# Autodesk Inventor assembly: 20-J2
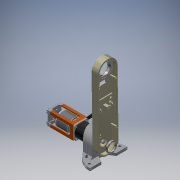
[picture p0: Inventor's stored thumbnail of the model, 180x180]
Saved by Autodesk Inventor 2018 (Build 220112000, 112)
## iProperties
Created: 2020-01-14
Part Number: 20-J2
Document SubType Name: Assembly
Designer: Bunny320
Author: Bunny320
## Documents named in this file (10)
- C:\Users\Bunny320\Desktop\sechs\4-CAD\30-J3.iam
- C:\Users\Bunny320\Desktop\sechs\4-CAD\201-flange-with motor.ipt
- C:\Users\Bunny320\Desktop\sechs\4-CAD\standardParts\61807-2RS1\61807-2RS1.iam
- C:\Users\Bunny320\Desktop\sechs\4-CAD\motor unit.iam
- C:\Users\Bunny320\Desktop\sechs\4-CAD\303-link right.ipt
- C:\Users\Bunny320\Desktop\sechs\4-CAD\generated\J3_belt.iam
- C:\Users\Bunny320\Desktop\sechs\4-CAD\standardParts\61705-2RZ\W 61705-2RZ.iam
- C:\Users\Bunny320\Desktop\sechs\4-CAD\standardParts\W 638_3-2Z\W 638_3-2Z.iam
- C:\Users\Bunny320\Documents\Inventor\Content Center Files\R2018\en-US\ISO 10642(2)\ISO 10642  - M4  x  20.ipt
- C:\Users\Bunny320\Documents\Inventor\Content Center Files\R2018\en-US\ISO 4762(1)\DIN EN ISO 4762 - M3 x 12.ipt
## Components (15 placed, 9 different names)
1. 201-flange-with motor:1 — Flush:1, Flush:2, Flush:3, Mate:3, Mate:4, Mate:7, Mate:8, Mate:9, Mate:22, Mate:23, Mate:24, Mate:25
2. 61807-2RS1:1 [sub-assembly] — Mate:3, Mate:4, Mate:10, Mate:11
3. 61807-2RS1:2 [sub-assembly] — Mate:12, Mate:13
4. motor unit:1 [sub-assembly] — Mate:7, Mate:8, Mate:9, Mate:14
5. 303-link right:1 — Mate:10, Mate:11, Mate:12, Mate:13, Flush:4, Mate:17, Mate:18, Mate:19, Mate:20, Mate:21, Mate:26, Mate:32
6. J3_belt:1 [sub-assembly] — Flush:4, Mate:14, Mate:15, Mate:16, Mate:17
7. W 61705-2RZ:1 [sub-assembly] — Mate:15, Mate:16
8. W 638_3-2Z:1 [sub-assembly] — Mate:18, Mate:21, Mate:27, Mate:33
9. W 638_3-2Z:2 [sub-assembly] — Mate:19, Mate:20
10. DIN EN ISO 10642 M4  x  20:1 — Mate:22
11. DIN EN ISO 10642 M4  x  20:2 — Mate:23
12. DIN EN ISO 10642 M4  x  20:3 — Mate:24
13. DIN EN ISO 10642 M4  x  20:4 — Mate:25
14. DIN EN ISO 4762 M3 x 12:1 — Mate:26, Mate:27
15. DIN EN ISO 4762 M3 x 12:4 — Mate:32, Mate:33
## Relationships (29: Mate 25, Flush 4)
- Flush:1: 201-flange-with motor:1
- Flush:2: 201-flange-with motor:1
- Flush:3: 201-flange-with motor:1
- Mate:3: 201-flange-with motor:1 ↔ 61807-2RS1:1
- Mate:4: 201-flange-with motor:1 ↔ 61807-2RS1:1
- Mate:7: 201-flange-with motor:1 ↔ motor unit:1
- Mate:8: 201-flange-with motor:1 ↔ motor unit:1
- Mate:9: 201-flange-with motor:1 ↔ motor unit:1
- Mate:10: 61807-2RS1:1 ↔ 303-link right:1
- Mate:11: 61807-2RS1:1 ↔ 303-link right:1
- Mate:12: 61807-2RS1:2 ↔ 303-link right:1
- Mate:13: 61807-2RS1:2 ↔ 303-link right:1
- Flush:4: 303-link right:1 ↔ J3_belt:1
- Mate:14: motor unit:1 ↔ J3_belt:1
- Mate:15: J3_belt:1 ↔ W 61705-2RZ:1
- Mate:16: J3_belt:1 ↔ W 61705-2RZ:1
- Mate:17: 303-link right:1 ↔ J3_belt:1
- Mate:18: 303-link right:1 ↔ W 638_3-2Z:1
- Mate:19: 303-link right:1 ↔ W 638_3-2Z:2
- Mate:20: 303-link right:1 ↔ W 638_3-2Z:2
- Mate:21: 303-link right:1 ↔ W 638_3-2Z:1
- Mate:22: 201-flange-with motor:1 ↔ DIN EN ISO 10642 M4  x  20:1
- Mate:23: 201-flange-with motor:1 ↔ DIN EN ISO 10642 M4  x  20:2
- Mate:24: 201-flange-with motor:1 ↔ DIN EN ISO 10642 M4  x  20:3
- Mate:25: 201-flange-with motor:1 ↔ DIN EN ISO 10642 M4  x  20:4
- Mate:26: 303-link right:1 ↔ DIN EN ISO 4762 M3 x 12:1
- Mate:27: W 638_3-2Z:1 ↔ DIN EN ISO 4762 M3 x 12:1
- Mate:32: 303-link right:1 ↔ DIN EN ISO 4762 M3 x 12:4
- Mate:33: W 638_3-2Z:1 ↔ DIN EN ISO 4762 M3 x 12:4
